# Autodesk Inventor assembly: conveyour 3
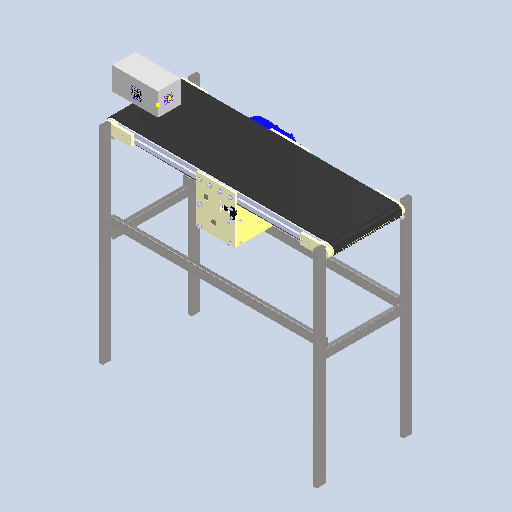
[picture p0: Inventor's stored thumbnail of the model, 512x512]
Saved by Autodesk Inventor 2022.2 (Build 262287000, 287)
## iProperties
Created: 2022-02-23
Part Number: conveyour 3
Document SubType Name: Assembly
Designer: ONG
Author: ONG
## Documents named in this file (6)
- C:\Users\ONG\Documents\INVENTOR DESIGN\音箱\conveyour 3.iam
- C:\Users\ONG\Downloads\belt conveyour\ARCANE 300х1000\Frame\Frame 1645576523614.iam
- C:\Users\ONG\Downloads\belt conveyour\ARCANE 300х1000.iam
- C:\Users\ONG\Documents\INVENTOR DESIGN\音箱\stand one part.ipt
- C:\Users\ONG\Documents\INVENTOR DESIGN\音箱\total asssembly\Frame\Frame 1645577982344.iam
- C:\Users\ONG\Documents\INVENTOR DESIGN\音箱\OBJECT.ipt
## Components (8 placed, 5 different names)
1. Frame 1645576523614:1 [sub-assembly]
2. ARCANE 300х1000:1 [sub-assembly]
3. stand one part:1
4. stand one part:2
5. stand one part:3
6. stand one part:4
7. Frame 1645577982344:1 [sub-assembly]
8. OBJECT:1
## Relationships (15: Mate 9, Flush 5, WeldJoint 1)
- [Mate]: Frame 1645576523614:1 ↔ ARCANE 300х1000:1
- [Mate]: Frame 1645576523614:1 ↔ stand one part:3
- [Flush] (-5 mm): Frame 1645576523614:1 ↔ stand one part:4
- [Mate]: Frame 1645576523614:1 ↔ stand one part:4
- [Mate]: stand one part:3 ↔ Frame 1645577982344:1
- [Flush]: stand one part:3 ↔ Frame 1645577982344:1
- [Mate]: stand one part:4 ↔ Frame 1645577982344:1
- [Flush]: stand one part:2 ↔ Frame 1645577982344:1
- [Mate]: stand one part:2 ↔ Frame 1645577982344:1
- [Mate]: Frame 1645576523614:1 ↔ stand one part:2
- [Flush]: stand one part:1 ↔ Frame 1645577982344:1
- [Mate]: Frame 1645576523614:1 ↔ stand one part:1
- [Mate]: stand one part:1 ↔ Frame 1645577982344:1
- [Flush]: Frame 1645576523614:1 ↔ Frame 1645577982344:1
- [WeldJoint]: ARCANE 300х1000:1 ↔ OBJECT:1
## Named parameters: d2_d10 = 0 mm, d3_d11 = -5 mm, d4_d12 = 0 mm, d5_d14 = 0 mm, d6_d15 = 0 mm, d7_d16 = 0 mm, d8_d17 = 0 mm
